# Autodesk Inventor assembly: thicc
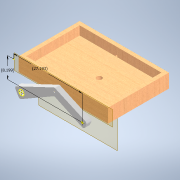
[picture p0: Inventor's stored thumbnail of the model, 180x180]
Saved by Autodesk Inventor 2020 (Build 240168000, 168)
## iProperties
Created: 2020-08-04
Part Number: thicc
Document SubType Name: Assembly
Designer: Manish
Author: Manish
## Documents named in this file (4)
- C:\Users\Manish\Documents\inventor\thicc.iam
- C:\Users\Manish\Documents\inventor\Ref\basefresh.ipt
- C:\Users\Public\Documents\Autodesk\Inventor 2020\bogie1.ipt
- C:\Users\Public\Documents\Autodesk\Inventor 2020\boogie2.ipt
## Components (3 placed, 3 different names)
1. basefresh:1 — Flush:1, Flush:2, Rotation:1
2. bogie1:1 — Flush:1, Flush:2, Rotation:1
3. boogie2:1
## Relationships (3: Flush 2, RelateRotation 1)
- Flush:1: basefresh:1 ↔ bogie1:1
- Flush:2: basefresh:1 ↔ bogie1:1
- Rotation:1 [RelateRotation] (1 ul): basefresh:1 ↔ bogie1:1
